# Autodesk Inventor assembly: Stepper Motor
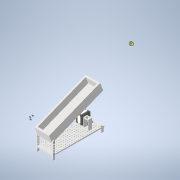
[picture p0: Inventor's stored thumbnail of the model, 180x180]
Saved by Autodesk Inventor 2021 (Build 250183000, 183)
## iProperties
Created: 2020-12-15
Part Number: Stepper Motor
Document SubType Name: Assembly
Designer: bestm
Author: bestm
## Documents named in this file (8)
- C:\Users\Yuvraj Sandhu\Desktop\Team14_P3_Milestone4 (Modelling)\Team 14 P3 Modelling Files\Stepper Motor.iam
- C:\Users\Yuvraj Sandhu\Desktop\Team14_P3_Milestone4 (Modelling)\Team 14 P3 Modelling Files\Stepper Motor Housing.ipt
- C:\Users\Yuvraj Sandhu\Desktop\Team14_P3_Milestone4 (Modelling)\Team 14 P3 Modelling Files\Stepper Motor Axle.ipt
- C:\Users\Yuvraj Sandhu\Desktop\Team14_P3_Milestone4 (Modelling)\Team 14 P3 Modelling Files\Mounting Platform.iam
- C:\Users\Yuvraj Sandhu\Desktop\Team14_P3_Milestone4 (Modelling)\Team 14 P3 Modelling Files\GivenHopper (to be modified by your team).ipt
- C:\Users\Yuvraj Sandhu\Desktop\Team14_P3_Milestone4 (Modelling)\Team 14 P3 Modelling Files\Short Screw (Stepper Motor & Linear Actuator).ipt
- C:\Users\Yuvraj Sandhu\Desktop\Team14_P3_Milestone4 (Modelling)\Team 14 P3 Modelling Files\Part2.ipt
- C:\Users\Yuvraj Sandhu\Desktop\Team14_P3_Milestone4 (Modelling)\Team 14 P3 Modelling Files\Spur Gears3.iam
## Components (20 placed, 7 different names)
1. Stepper Motor Housing:1 — Mate:1, Mate:2, Mate:3, Mate:4, Mate:5, Insert:3, Insert:4, Insert:5
2. Stepper Motor Axle:1 — Mate:1, Mate:2, Mate:10, Insert:11
3. Mounting Platform:1 [sub-assembly] — Mate:3, Mate:4, Mate:5, Mate:6, Mate:7, Mate:8, Insert:1, Insert:2, Mate:9, Insert:6, Insert:7, Insert:8, Insert:9, Insert:10
4. GivenHopper (to be modified by your team):1 — Mate:6, Mate:7, Mate:8
5. Short Screw (Stepper Motor & Linear Actuator):1 — Insert:4
6. Short Screw (Stepper Motor & Linear Actuator):2 — Insert:5
7. Short Screw (Stepper Motor & Linear Actuator):3 — Insert:3
8. Short Screw (Stepper Motor & Linear Actuator):4 — Insert:2
9. Short Screw (Stepper Motor & Linear Actuator):5 — Insert:1
10. Part2:1 — Mate:9
11. Spur Gears:2 [sub-assembly] — Mate:10, Insert:11
12. Short Screw (Stepper Motor & Linear Actuator):6 — Insert:9
13. Short Screw (Stepper Motor & Linear Actuator):7 — Insert:8
14. Short Screw (Stepper Motor & Linear Actuator):8 — Insert:7
15. Short Screw (Stepper Motor & Linear Actuator):9 — Insert:10
16. Short Screw (Stepper Motor & Linear Actuator):10 — Insert:6
17. Short Screw (Stepper Motor & Linear Actuator):11
18. Short Screw (Stepper Motor & Linear Actuator):12
19. Short Screw (Stepper Motor & Linear Actuator):13
20. Short Screw (Stepper Motor & Linear Actuator):14
## Relationships (21: Insert 11, Mate 10)
- Mate:1: Stepper Motor Housing:1 ↔ Stepper Motor Axle:1
- Mate:2: Stepper Motor Housing:1 ↔ Stepper Motor Axle:1
- Mate:3: Stepper Motor Housing:1 ↔ Mounting Platform:1
- Mate:4: Stepper Motor Housing:1 ↔ Mounting Platform:1
- Mate:5: Stepper Motor Housing:1 ↔ Mounting Platform:1
- Mate:6: Mounting Platform:1 ↔ GivenHopper (to be modified by your team):1
- Mate:7: Mounting Platform:1 ↔ GivenHopper (to be modified by your team):1
- Mate:8: Mounting Platform:1 ↔ GivenHopper (to be modified by your team):1
- Insert:1: Mounting Platform:1 ↔ Short Screw (Stepper Motor & Linear Actuator):5
- Insert:2: Mounting Platform:1 ↔ Short Screw (Stepper Motor & Linear Actuator):4
- Insert:3: Stepper Motor Housing:1 ↔ Short Screw (Stepper Motor & Linear Actuator):3
- Insert:4: Stepper Motor Housing:1 ↔ Short Screw (Stepper Motor & Linear Actuator):1
- Insert:5: Stepper Motor Housing:1 ↔ Short Screw (Stepper Motor & Linear Actuator):2
- Mate:9: Mounting Platform:1 ↔ Part2:1
- Insert:6: Mounting Platform:1 ↔ Short Screw (Stepper Motor & Linear Actuator):10
- Insert:7: Mounting Platform:1 ↔ Short Screw (Stepper Motor & Linear Actuator):8
- Insert:8: Mounting Platform:1 ↔ Short Screw (Stepper Motor & Linear Actuator):7
- Insert:9: Mounting Platform:1 ↔ Short Screw (Stepper Motor & Linear Actuator):6
- Insert:10: Mounting Platform:1 ↔ Short Screw (Stepper Motor & Linear Actuator):9
- Mate:10: Stepper Motor Axle:1 ↔ Spur Gears:2
- Insert:11 (-5.5 mm): Stepper Motor Axle:1 ↔ Spur Gears:2
